# Autodesk Inventor assembly: Kolo
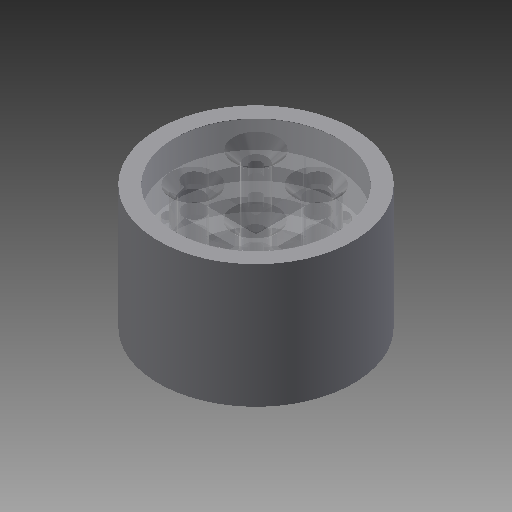
[picture p0: Inventor's stored thumbnail of the model, 512x512]
Saved by Autodesk Inventor 2019 (Build 230136000, 136)
## iProperties
Created: 2022-03-19
Part Number: Kolo
Material: Ogólny
Document SubType Name: Assembly
Designer: Michał
Author: Michał
## Documents named in this file (3)
- D:\Projekty\Roboty\Karzel\3D\3D\Kolo.iam
- D:\Projekty\Roboty\Karzel\3D\3D\Felga.ipt
- D:\Projekty\Roboty\Karzel\3D\3D\Opona.ipt
## Components (2 placed, 2 different names)
1. Felga:1 — Zestawiający:1, Równoległy:1
2. Opona:1 — Zestawiający:1, Równoległy:1
## Relationships (2: Mate 1, Flush 1)
- Zestawiający:1 [Mate]: Felga:1 ↔ Opona:1
- Równoległy:1 [Flush]: Felga:1 ↔ Opona:1
